# Autodesk Inventor assembly: actuator_MIR
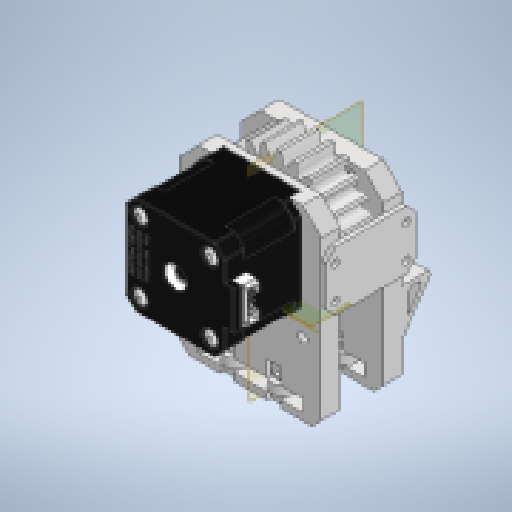
[picture p0: Inventor's stored thumbnail of the model, 512x512]
Saved by Autodesk Inventor 2023.1 (Build 271208000, 208)
## iProperties
Created: 2025-12-13
Part Number: actuator_MIR
Document SubType Name: Assembly
Designer: DELL
Author: DELL
## Documents named in this file (9)
- C:\Users\DELL\reposGitHub\VSOSH25-26\models\actuator\actuator_MIR.iam
- C:\Users\DELL\reposGitHub\VSOSH25-26\models\import\Schrittmotor-42SHDC3025-24B_MIR.ipt
- C:\Users\DELL\reposGitHub\VSOSH25-26\models\actuator\звезда_шестрерни_MIR.ipt
- C:\Users\DELL\reposGitHub\VSOSH25-26\models\actuator\муфта_MIR.ipt
- C:\Users\DELL\reposGitHub\VSOSH25-26\models\actuator\шестреня_12.12_MIR.ipt
- C:\Users\DELL\reposGitHub\VSOSH25-26\models\actuator\каретка_MIR.ipt
- C:\Users\DELL\reposGitHub\VSOSH25-26\models\actuator\колесико_MIR.ipt
- C:\Users\DELL\reposGitHub\VSOSH25-26\models\actuator\стена_простая_MIR.ipt
- C:\Users\DELL\reposGitHub\VSOSH25-26\models\actuator\каретка_м3_без_м_MIR.ipt
## Components (11 placed, 8 different names)
1. Schrittmotor-42SHDC3025-24B_MIR:1 — Совмещение:2, Совмещение:1, Заподлицо:1, Совмещение:4, Заподлицо:3
2. звезда_шестрерни_MIR:1 — Совмещение:6, Совмещение:5, Заподлицо:2, Совмещение:8, Совмещение:7
3. муфта_MIR:1 — Совмещение:6, Совмещение:5, Совмещение:4, Совмещение:9
4. шестреня_12.12_MIR:1 — Заподлицо:2, Совмещение:8, Совмещение:7
5. каретка_MIR:1 — Совмещение:9, Заподлицо:3, Совмещение:53, Совмещение:43, Совмещение:37, Совмещение:52, Совмещение:41, Заподлицо:5, Совмещение:61
6. колесико_MIR:1 — Совмещение:53, Совмещение:43
7. стена_простая_MIR:1 — Совмещение:37
8. колесико_MIR:2 — Совмещение:52, Совмещение:41
9. каретка_м3_без_м_MIR:1 — Заподлицо:5, Совмещение:61, Совмещение:60, Совмещение:59, Совмещение:58, Совмещение:57
10. колесико_MIR:3 — Совмещение:60, Совмещение:59
11. колесико_MIR:4 — Совмещение:58, Совмещение:57
## Relationships (22: Mate 20, Flush 2)
- Совмещение:2 [Mate]: Schrittmotor-42SHDC3025-24B_MIR:1
- Совмещение:1 [Mate]: Schrittmotor-42SHDC3025-24B_MIR:1
- Заподлицо:1 [Mate]: Schrittmotor-42SHDC3025-24B_MIR:1
- Совмещение:6 [Mate]: звезда_шестрерни_MIR:1 ↔ муфта_MIR:1
- Совмещение:5 [Mate]: звезда_шестрерни_MIR:1 ↔ муфта_MIR:1
- Совмещение:4 [Mate]: Schrittmotor-42SHDC3025-24B_MIR:1 ↔ муфта_MIR:1
- Заподлицо:2 [Flush]: звезда_шестрерни_MIR:1 ↔ шестреня_12.12_MIR:1
- Совмещение:8 [Mate]: звезда_шестрерни_MIR:1 ↔ шестреня_12.12_MIR:1
- Совмещение:7 [Mate]: звезда_шестрерни_MIR:1 ↔ шестреня_12.12_MIR:1
- Совмещение:9 [Mate] (0.5 mm): муфта_MIR:1 ↔ каретка_MIR:1
- Заподлицо:3 [Mate]: Schrittmotor-42SHDC3025-24B_MIR:1 ↔ каретка_MIR:1
- Совмещение:53 [Mate]: каретка_MIR:1 ↔ колесико_MIR:1
- Совмещение:43 [Mate]: каретка_MIR:1 ↔ колесико_MIR:1
- Совмещение:37 [Mate]: каретка_MIR:1 ↔ стена_простая_MIR:1
- Совмещение:52 [Mate]: каретка_MIR:1 ↔ колесико_MIR:2
- Совмещение:41 [Mate]: каретка_MIR:1 ↔ колесико_MIR:2
- Заподлицо:5 [Flush]: каретка_MIR:1 ↔ каретка_м3_без_м_MIR:1
- Совмещение:61 [Mate] (18.2 mm): каретка_MIR:1 ↔ каретка_м3_без_м_MIR:1
- Совмещение:60 [Mate]: каретка_м3_без_м_MIR:1 ↔ колесико_MIR:3
- Совмещение:59 [Mate]: каретка_м3_без_м_MIR:1 ↔ колесико_MIR:3
- Совмещение:58 [Mate]: каретка_м3_без_м_MIR:1 ↔ колесико_MIR:4
- Совмещение:57 [Mate]: каретка_м3_без_м_MIR:1 ↔ колесико_MIR:4
